# Autodesk Inventor assembly: FinalRobot-ver13-1111-2021
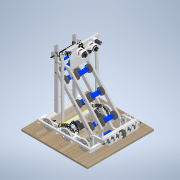
[picture p0: Inventor's stored thumbnail of the model, 180x180]
Saved by Autodesk Inventor 2021 (Build 250183000, 183)
## iProperties
Created: 2021-01-26
Part Number: FinalRobot-ver13-1111-2021
Document SubType Name: Assembly
Designer: Caitlin
Author: Caitlin
## Documents named in this file (6)
- C:\Users\con_c_000\Documents\GitHub\RoboticsCad1111\PHRC CADD\2020 Infinite Recharge\2021 Infinite Recharge\FinalRobot-ver13-1111-2021.iam
- C:\Users\con_c_000\Documents\GitHub\RoboticsCad1111\PHRC CADD\2020 Infinite Recharge\2021 Infinite Recharge\Chassis\Chassis-ver1-1111-2021.iam
- C:\Users\con_c_000\Documents\GitHub\RoboticsCad1111\PHRC CADD\2020 Infinite Recharge\Platform.ver1-1111-2020.ipt
- C:\Users\con_c_000\Documents\GitHub\RoboticsCad1111\PHRC CADD\2020 Infinite Recharge\2021 Infinite Recharge\Chassis\Shooter-Storage-IntakeAssembly.ver4-1111-2021.iam
- C:\Users\con_c_000\Documents\GitHub\RoboticsCad1111\PHRC CADD\2020 Infinite Recharge\2021 Infinite Recharge\Chassis\PnumaticActiveClimb-ver3-1111-2021.iam
- C:\Users\con_c_000\Documents\GitHub\RoboticsCad1111\PHRC CADD\Resources\VEXpro Resources\Wheels\Wheel Parts\6_ Traction Tire - 0.5_ Wide (217-2860).iam
## Components (10 placed, 5 different names)
1. Chassis-ver1-1111-2021:1 [sub-assembly] — Mate:1, Angle:1, Flush:1, Flush:2, Mate:2, Mate:3, Flush:3, Mate:4, Flush:4, Flush:5, Mate:5, Mate:6, Mate:7, Mate:8, Mate:9, Mate:10, Mate:11, Mate:12, Mate:13, Mate:14, Mate:15, Mate:16, Mate:17, Mate:18, Mate:19, Mate:20, Mate:21, Mate:22
2. Platform.ver1-1111-2020:1 — Mate:1, Angle:1, Flush:1, Flush:2
3. Shooter-Storage-IntakeAssembly.ver4-1111-2021:1 [sub-assembly] — Mate:2, Mate:3, Flush:3
4. PnumaticActiveClimb-ver3-1111-2021:1 [sub-assembly] — Mate:4, Flush:4, Flush:5
5. 6_ Traction Tire - 0.5_ Wide (217-2860):1 [sub-assembly] — Mate:11, Mate:12, Mate:13
6. 6_ Traction Tire - 0.5_ Wide (217-2860):2 [sub-assembly] — Mate:8, Mate:9, Mate:10
7. 6_ Traction Tire - 0.5_ Wide (217-2860):3 [sub-assembly] — Mate:5, Mate:6, Mate:7
8. 6_ Traction Tire - 0.5_ Wide (217-2860):4 [sub-assembly] — Mate:14, Mate:15, Mate:16
9. 6_ Traction Tire - 0.5_ Wide (217-2860):5 [sub-assembly] — Mate:17, Mate:18, Mate:19
10. 6_ Traction Tire - 0.5_ Wide (217-2860):6 [sub-assembly] — Mate:20, Mate:21, Mate:22
## Relationships (28: Mate 22, Flush 5, Angle 1)
- Mate:1 (47.625 mm): Chassis-ver1-1111-2021:1 ↔ Platform.ver1-1111-2020:1
- Angle:1 (0 deg): Chassis-ver1-1111-2021:1 ↔ Platform.ver1-1111-2020:1
- Flush:1 (152.4 mm): Chassis-ver1-1111-2021:1 ↔ Platform.ver1-1111-2020:1
- Flush:2 (114.3 mm): Chassis-ver1-1111-2021:1 ↔ Platform.ver1-1111-2020:1
- Mate:2: Chassis-ver1-1111-2021:1 ↔ Shooter-Storage-IntakeAssembly.ver4-1111-2021:1
- Mate:3: Chassis-ver1-1111-2021:1 ↔ Shooter-Storage-IntakeAssembly.ver4-1111-2021:1
- Flush:3: Chassis-ver1-1111-2021:1 ↔ Shooter-Storage-IntakeAssembly.ver4-1111-2021:1
- Mate:4: Chassis-ver1-1111-2021:1 ↔ PnumaticActiveClimb-ver3-1111-2021:1
- Flush:4: Chassis-ver1-1111-2021:1 ↔ PnumaticActiveClimb-ver3-1111-2021:1
- Flush:5: Chassis-ver1-1111-2021:1 ↔ PnumaticActiveClimb-ver3-1111-2021:1
- Mate:5: Chassis-ver1-1111-2021:1 ↔ 6_ Traction Tire - 0.5_ Wide (217-2860):3
- Mate:6: Chassis-ver1-1111-2021:1 ↔ 6_ Traction Tire - 0.5_ Wide (217-2860):3
- Mate:7: Chassis-ver1-1111-2021:1 ↔ 6_ Traction Tire - 0.5_ Wide (217-2860):3
- Mate:8: Chassis-ver1-1111-2021:1 ↔ 6_ Traction Tire - 0.5_ Wide (217-2860):2
- Mate:9: Chassis-ver1-1111-2021:1 ↔ 6_ Traction Tire - 0.5_ Wide (217-2860):2
- Mate:10: Chassis-ver1-1111-2021:1 ↔ 6_ Traction Tire - 0.5_ Wide (217-2860):2
- Mate:11: Chassis-ver1-1111-2021:1 ↔ 6_ Traction Tire - 0.5_ Wide (217-2860):1
- Mate:12: Chassis-ver1-1111-2021:1 ↔ 6_ Traction Tire - 0.5_ Wide (217-2860):1
- Mate:13: Chassis-ver1-1111-2021:1 ↔ 6_ Traction Tire - 0.5_ Wide (217-2860):1
- Mate:14: Chassis-ver1-1111-2021:1 ↔ 6_ Traction Tire - 0.5_ Wide (217-2860):4
- Mate:15: Chassis-ver1-1111-2021:1 ↔ 6_ Traction Tire - 0.5_ Wide (217-2860):4
- Mate:16: Chassis-ver1-1111-2021:1 ↔ 6_ Traction Tire - 0.5_ Wide (217-2860):4
- Mate:17: Chassis-ver1-1111-2021:1 ↔ 6_ Traction Tire - 0.5_ Wide (217-2860):5
- Mate:18: Chassis-ver1-1111-2021:1 ↔ 6_ Traction Tire - 0.5_ Wide (217-2860):5
- Mate:19: Chassis-ver1-1111-2021:1 ↔ 6_ Traction Tire - 0.5_ Wide (217-2860):5
- Mate:20: Chassis-ver1-1111-2021:1 ↔ 6_ Traction Tire - 0.5_ Wide (217-2860):6
- Mate:21: Chassis-ver1-1111-2021:1 ↔ 6_ Traction Tire - 0.5_ Wide (217-2860):6
- Mate:22: Chassis-ver1-1111-2021:1 ↔ 6_ Traction Tire - 0.5_ Wide (217-2860):6
